# Autodesk Inventor assembly: Gripper
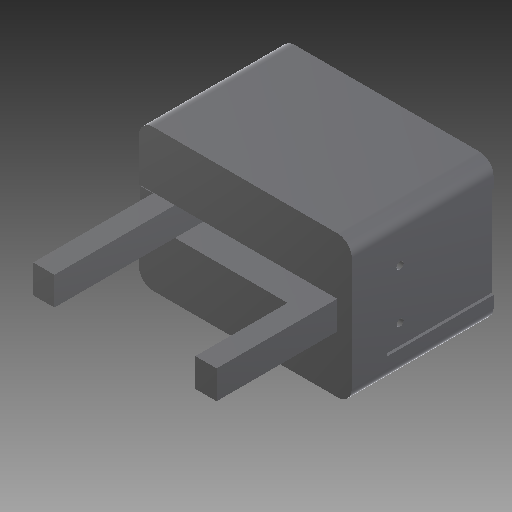
[picture p0: Inventor's stored thumbnail of the model, 512x512]
Saved by Autodesk Inventor 2017 (Build 210142000, 142)
## iProperties
Created: 2018-10-23
Part Number: Gripper
Document SubType Name: Assembly
Designer: Dell
Author: Dell
## Documents named in this file (6)
- C:\Users\Dell\Documents\GitHub\tr2\Gripper\Gripper.iam
- C:\Users\Dell\Documents\GitHub\tr2\Gripper\GA01.ipt
- C:\Users\Dell\Documents\GitHub\tr2\Gripper\AX-12A.ipt
- C:\Users\Dell\Documents\GitHub\tr2\Gripper\GA03.ipt
- C:\Users\Dell\Documents\GitHub\tr2\Gripper\Gripper\Design Accelerator\Spur Gears1.iam
- C:\Users\Dell\Documents\GitHub\tr2\Gripper\GA04.ipt
## Components (6 placed, 5 different names)
1. GA01:1 — Mate:8, Mate:9, Mate:10, Mate:11, Mate:12, Mate:17, Mate:19
2. GA03:1 — Mate:10, Mate:11, Mate:12, Mate:13, Mate:14, Mate:20
3. AX-12A:1 — Mate:8, Mate:9, Mate:13, Mate:14, Mate:15, Mate:16, Mate:20
4. Spur Gears:1 [sub-assembly] — Mate:15, Mate:16, Rotation/Translation:1, Rotation/Translation:2, Flush:1, Flush:2
5. GA04:1 — Mate:17, Rotation/Translation:1, Flush:2
6. GA04:2 — Mate:19, Rotation/Translation:2, Flush:1
## Relationships (16: Mate 12, RelateRotateTranslate 2, Flush 2)
- Mate:8: GA01:1 ↔ AX-12A:1
- Mate:9: GA01:1 ↔ AX-12A:1
- Mate:10: GA01:1 ↔ GA03:1
- Mate:11: GA01:1 ↔ GA03:1
- Mate:12: GA01:1 ↔ GA03:1
- Mate:13: GA03:1 ↔ AX-12A:1
- Mate:14: GA03:1 ↔ AX-12A:1
- Mate:15: AX-12A:1 ↔ Spur Gears:1
- Mate:16: AX-12A:1 ↔ Spur Gears:1
- Mate:17: GA01:1 ↔ GA04:1
- Mate:19: GA01:1 ↔ GA04:2
- Rotation/Translation:1 [RelateRotateTranslate] (131 mm): Spur Gears:1 ↔ GA04:1
- Rotation/Translation:2 [RelateRotateTranslate] (131 mm): Spur Gears:1 ↔ GA04:2
- Mate:20: GA03:1 ↔ AX-12A:1
- Flush:1: Spur Gears:1 ↔ GA04:2
- Flush:2: Spur Gears:1 ↔ GA04:1
